# Autodesk Inventor assembly: RobotPrototype
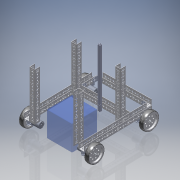
[picture p0: Inventor's stored thumbnail of the model, 180x180]
Saved by Autodesk Inventor 2017 (Build 210142000, 142)
## iProperties
Created: 2017-09-10
Part Number: RobotPrototype
Document SubType Name: Assembly
Designer: Kenneth
Author: Kenneth
## Documents named in this file (10)
- C:\Workspaces\CAD\RobotPrototype.iam
- C:\Users\Public\Documents\Autodesk\Inventor 2017\Spectrum-CAD-Library\FTC\FTC Tetrix KOP\Channel 416mm.ipt
- C:\Users\Public\Documents\Autodesk\Inventor 2017\Spectrum-CAD-Library\FTC\FTC Tetrix KOP\Bracket L-angle.ipt
- C:\Users\Public\Documents\Autodesk\Inventor 2017\Spectrum-CAD-Library\FTC\FTC Tetrix KOP\Channel 288mm.ipt
- C:\Users\Public\Documents\Autodesk\Inventor 2017\Spectrum-CAD-Library\FTC\FTC Tetrix KOP\DC Motor Mount.ipt
- C:\Users\Public\Documents\Autodesk\Inventor 2017\Spectrum-CAD-Library\FTC\FTC Tetrix KOP\DC Gearhead Motor.ipt
- C:\Users\Public\Documents\Autodesk\Inventor 2017\Spectrum-CAD-Library\FTC\FTC Tetrix KOP\Axle Shaft Hub.ipt
- C:\Users\Public\Documents\Autodesk\Inventor 2017\Spectrum-CAD-Library\FTC\FTC Tetrix KOP\Wheel 101.6mm (4in).ipt
- C:\Users\Public\Documents\Autodesk\Inventor 2017\Glyph.ipt
- C:\Users\Public\Documents\Autodesk\Inventor 2017\15mm Extrusion REV-41-1017.ipt
## Components (30 placed, 9 different names)
1. Channel 416mm:1 — Mate:3, Mate:4, Mate:12, Mate:24, Mate:34, Mate:35, Mate:36, Mate:37, Mate:38, Mate:39, Mate:69, Mate:70, Mate:71, Mate:75, Mate:76, Mate:79, Mate:80, Mate:81, Mate:82
2. Channel 416mm:2 — Mate:7, Mate:8, Mate:9, Mate:21, Mate:29, Mate:30, Mate:31, Mate:32, Mate:33, Mate:65, Mate:72, Mate:73, Mate:74, Mate:77, Mate:78, Mate:83, Mate:84, Mate:85
3. Bracket L-angle:1 — Mate:69, Mate:70, Mate:71
4. Bracket L-angle:3 — Mate:3, Mate:4, Mate:12, Mate:13, Mate:14, Mate:23, Mate:24
5. Bracket L-angle:4 — Mate:7, Mate:8, Mate:9, Mate:15, Mate:16, Mate:21, Mate:22
6. Channel 288mm:1 — Mate:13, Mate:14, Mate:15, Mate:16, Mate:22, Mate:23
7. Channel 288mm:2 — Mate:86, Mate:87, Angle:1
8. DC Motor Mount:4 — Mate:29, Mate:30, Mate:31, Mate:42, Flush:6
9. DC Motor Mount:5 — Mate:32, Mate:33, Mate:43, Flush:5, Mate:65
10. DC Motor Mount:6 — Mate:34, Mate:35, Mate:36, Mate:40, Mate:41, Flush:7
11. DC Motor Mount:7 — Mate:37, Mate:38, Mate:39, Mate:44, Flush:8
12. DC Gearhead Motor:1 — Mate:40, Mate:41, Mate:46, Mate:52, Mate:57, Flush:7
13. DC Gearhead Motor:2 — Mate:44, Mate:45, Mate:51, Mate:58, Flush:8
14. DC Gearhead Motor:3 — Mate:42, Mate:49, Mate:50, Mate:60, Flush:6
15. DC Gearhead Motor:4 — Mate:43, Mate:47, Mate:48, Mate:59, Flush:5
16. Axle Shaft Hub:1 — Mate:45, Mate:51, Mate:55, Mate:64
17. Axle Shaft Hub:2 — Mate:47, Mate:48, Mate:54, Mate:62
18. Axle Shaft Hub:3 — Mate:49, Mate:50, Mate:53, Mate:61
19. Axle Shaft Hub:4 — Mate:46, Mate:52, Mate:56, Mate:63
20. Wheel 101.6mm (4in):1 — Mate:56, Mate:57, Mate:63
21. Wheel 101.6mm (4in):2 — Mate:55, Mate:58, Mate:64
22. Wheel 101.6mm (4in):3 — Mate:54, Mate:59, Mate:62
23. Wheel 101.6mm (4in):4 — Mate:53, Mate:60, Mate:61
24. Bracket L-angle:5 — Mate:72, Mate:73
25. Glyph:1
26. Channel 288mm:3 — Mate:75, Mate:76, Mate:79
27. Channel 288mm:4 — Mate:74, Mate:77, Mate:78
28. Channel 288mm:5 — Mate:80, Mate:81, Mate:82
29. Channel 288mm:6 — Mate:83, Mate:84, Mate:85
30. 15mm Extrusion REV-41-1017:1 — Mate:86, Mate:87, Angle:1
## Relationships (75: Mate 70, Flush 4, Angle 1)
- Mate:3: Channel 416mm:1 ↔ Bracket L-angle:3
- Mate:4: Channel 416mm:1 ↔ Bracket L-angle:3
- Mate:7: Channel 416mm:2 ↔ Bracket L-angle:4
- Mate:8: Channel 416mm:2 ↔ Bracket L-angle:4
- Mate:9: Channel 416mm:2 ↔ Bracket L-angle:4
- Mate:12: Channel 416mm:1 ↔ Bracket L-angle:3
- Mate:13: Bracket L-angle:3 ↔ Channel 288mm:1
- Mate:14: Bracket L-angle:3 ↔ Channel 288mm:1
- Mate:15: Bracket L-angle:4 ↔ Channel 288mm:1
- Mate:16: Bracket L-angle:4 ↔ Channel 288mm:1
- Mate:21: Channel 416mm:2 ↔ Bracket L-angle:4
- Mate:22: Bracket L-angle:4 ↔ Channel 288mm:1
- Mate:23: Bracket L-angle:3 ↔ Channel 288mm:1
- Mate:24: Channel 416mm:1 ↔ Bracket L-angle:3
- Mate:29: Channel 416mm:2 ↔ DC Motor Mount:4
- Mate:30: Channel 416mm:2 ↔ DC Motor Mount:4
- Mate:31: Channel 416mm:2 ↔ DC Motor Mount:4
- Mate:32: Channel 416mm:2 ↔ DC Motor Mount:5
- Mate:33: Channel 416mm:2 ↔ DC Motor Mount:5
- Mate:34: Channel 416mm:1 ↔ DC Motor Mount:6
- Mate:35: Channel 416mm:1 ↔ DC Motor Mount:6
- Mate:36: Channel 416mm:1 ↔ DC Motor Mount:6
- Mate:37: Channel 416mm:1 ↔ DC Motor Mount:7
- Mate:38: Channel 416mm:1 ↔ DC Motor Mount:7
- Mate:39: Channel 416mm:1 ↔ DC Motor Mount:7
- Mate:40: DC Motor Mount:6 ↔ DC Gearhead Motor:1
- Mate:41: DC Motor Mount:6 ↔ DC Gearhead Motor:1
- Mate:42: DC Motor Mount:4 ↔ DC Gearhead Motor:3
- Mate:43: DC Motor Mount:5 ↔ DC Gearhead Motor:4
- Mate:44: DC Motor Mount:7 ↔ DC Gearhead Motor:2
- Mate:45: DC Gearhead Motor:2 ↔ Axle Shaft Hub:1
- Mate:46: DC Gearhead Motor:1 ↔ Axle Shaft Hub:4
- Mate:47: DC Gearhead Motor:4 ↔ Axle Shaft Hub:2
- Mate:48: DC Gearhead Motor:4 ↔ Axle Shaft Hub:2
- Mate:49: DC Gearhead Motor:3 ↔ Axle Shaft Hub:3
- Mate:50: DC Gearhead Motor:3 ↔ Axle Shaft Hub:3
- Mate:51: DC Gearhead Motor:2 ↔ Axle Shaft Hub:1
- Mate:52: DC Gearhead Motor:1 ↔ Axle Shaft Hub:4
- Mate:53: Axle Shaft Hub:3 ↔ Wheel 101.6mm (4in):4
- Mate:54: Axle Shaft Hub:2 ↔ Wheel 101.6mm (4in):3
- Mate:55: Axle Shaft Hub:1 ↔ Wheel 101.6mm (4in):2
- Mate:56: Axle Shaft Hub:4 ↔ Wheel 101.6mm (4in):1
- Mate:57: DC Gearhead Motor:1 ↔ Wheel 101.6mm (4in):1
- Mate:58: DC Gearhead Motor:2 ↔ Wheel 101.6mm (4in):2
- Mate:59: DC Gearhead Motor:4 ↔ Wheel 101.6mm (4in):3
- Mate:60: DC Gearhead Motor:3 ↔ Wheel 101.6mm (4in):4
- Mate:61: Axle Shaft Hub:3 ↔ Wheel 101.6mm (4in):4
- Mate:62: Axle Shaft Hub:2 ↔ Wheel 101.6mm (4in):3
- Mate:63: Axle Shaft Hub:4 ↔ Wheel 101.6mm (4in):1
- Mate:64: Axle Shaft Hub:1 ↔ Wheel 101.6mm (4in):2
- Flush:5: DC Motor Mount:5 ↔ DC Gearhead Motor:4
- Flush:6: DC Motor Mount:4 ↔ DC Gearhead Motor:3
- Flush:7: DC Motor Mount:6 ↔ DC Gearhead Motor:1
- Flush:8: DC Motor Mount:7 ↔ DC Gearhead Motor:2
- Mate:65: Channel 416mm:2 ↔ DC Motor Mount:5
- Mate:69: Channel 416mm:1 ↔ Bracket L-angle:1
- Mate:70: Channel 416mm:1 ↔ Bracket L-angle:1
- Mate:71: Channel 416mm:1 ↔ Bracket L-angle:1
- Mate:72: Channel 416mm:2 ↔ Bracket L-angle:5
- Mate:73: Channel 416mm:2 ↔ Bracket L-angle:5
- Mate:74: Channel 416mm:2 ↔ Channel 288mm:4
- Mate:75: Channel 416mm:1 ↔ Channel 288mm:3
- Mate:76: Channel 416mm:1 ↔ Channel 288mm:3
- Mate:77: Channel 416mm:2 ↔ Channel 288mm:4
- Mate:78: Channel 416mm:2 ↔ Channel 288mm:4
- Mate:79: Channel 416mm:1 ↔ Channel 288mm:3
- Mate:80: Channel 416mm:1 ↔ Channel 288mm:5
- Mate:81: Channel 416mm:1 ↔ Channel 288mm:5
- Mate:82: Channel 416mm:1 ↔ Channel 288mm:5
- Mate:83: Channel 416mm:2 ↔ Channel 288mm:6
- Mate:84: Channel 416mm:2 ↔ Channel 288mm:6
- Mate:85: Channel 416mm:2 ↔ Channel 288mm:6
- Mate:86: Channel 288mm:2 ↔ 15mm Extrusion REV-41-1017:1
- Mate:87: Channel 288mm:2 ↔ 15mm Extrusion REV-41-1017:1
- Angle:1 (90 deg): Channel 288mm:2 ↔ 15mm Extrusion REV-41-1017:1
